# Autodesk Inventor assembly: OpenRaman.V1
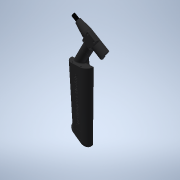
[picture p0: Inventor's stored thumbnail of the model, 180x180]
Saved by Autodesk Inventor 2020 (Build 240168000, 168)
## iProperties
Created: 2017-08-01
Part Number: OpenRaman.V1
Document SubType Name: Assembly
Designer: vmiguel
Author: vmiguel
## Documents named in this file (12)
- C:\Users\vmiguel\Documents\GitHub\OpenRaman\Hardware\OpenRaman.V1.iam
- C:\Users\vmiguel\Documents\GitHub\OpenRaman\Hardware\Supriments\TCD1304AP.ipt
- C:\Users\vmiguel\Documents\GitHub\OpenRaman\Hardware\PrismsGeometry.ipt
- C:\Users\vmiguel\Documents\GitHub\OpenRaman\Hardware\3D Printed Parts\SpectometerTube.ipt
- C:\Users\vmiguel\Documents\GitHub\OpenRaman\Hardware\3D Printed Parts\FirstPrismHolder.ipt
- C:\Users\vmiguel\Documents\GitHub\OpenRaman\Hardware\3D Printed Parts\PrismSensorHolder.ipt
- C:\Users\vmiguel\Documents\GitHub\OpenRaman\Hardware\Supriments\step_36396.ipt
- C:\Users\vmiguel\Documents\GitHub\OpenRaman\Hardware\Laser Cutted Parts\Slit.ipt
- C:\Users\vmiguel\Documents\GitHub\OpenRaman\Hardware\3D Printed Parts\NotchFilterScrew.ipt
- C:\Users\vmiguel\Documents\GitHub\OpenRaman\Hardware\3D Printed Parts\SpectoBoardCap.ipt
- C:\Users\vmiguel\Documents\GitHub\OpenRaman\Hardware\3D Printed Parts\RamanBody.ipt
- C:\Users\vmiguel\Documents\GitHub\OpenRaman\Hardware\Supriments\DPSSLaser.ipt
## Components (12 placed, 11 different names)
1. TCD1304AP:1 — Mate:3, Mate:4, Mate:5
2. PrismsGeometry:1 — Flush:2, Angle:1, Mate:1, Mate:2, Mate:3, Mate:4, Mate:5
3. SpectometerTube:1 — Flush:2, Angle:1, Mate:1, Flush:3, Flush:4
4. FirstPrismHolder:1 — Flush:3, Mate:2, Rotational:1, Mate:6, Mate:7, Flush:5, Rotational:3
5. PrismSensorHolder:1 — Flush:4, Flush:6
6. step_36396:1 — Rotational:1, Rotational:2
7. step_36396:2 — Rotational:2
8. Slit:1 — Mate:6, Mate:7
9. NotchFilterScrew:1 — Flush:5
10. SpectoBoardCap:1 — Flush:6
11. RamanBody:1 — Rotational:3, Rotational:4
12. DPSSLaser:1 — Rotational:4
## Relationships (17: Mate 7, Flush 5, RevoluteJoint 4, Angle 1)
- Flush:2: PrismsGeometry:1 ↔ SpectometerTube:1
- Angle:1 (-12 deg): PrismsGeometry:1 ↔ SpectometerTube:1
- Mate:1 (4 mm): PrismsGeometry:1 ↔ SpectometerTube:1
- Flush:3: SpectometerTube:1 ↔ FirstPrismHolder:1
- Mate:2: PrismsGeometry:1 ↔ FirstPrismHolder:1
- Mate:3: TCD1304AP:1 ↔ PrismsGeometry:1
- Mate:4: TCD1304AP:1 ↔ PrismsGeometry:1
- Mate:5: TCD1304AP:1 ↔ PrismsGeometry:1
- Flush:4: SpectometerTube:1 ↔ PrismSensorHolder:1
- Rotational:1 [RevoluteJoint]: FirstPrismHolder:1 ↔ step_36396:1
- Rotational:2 [RevoluteJoint] (15 mm): step_36396:1 ↔ step_36396:2
- Mate:6: FirstPrismHolder:1 ↔ Slit:1
- Mate:7: FirstPrismHolder:1 ↔ Slit:1
- Flush:5: FirstPrismHolder:1 ↔ NotchFilterScrew:1
- Flush:6: PrismSensorHolder:1 ↔ SpectoBoardCap:1
- Rotational:3 [RevoluteJoint]: FirstPrismHolder:1 ↔ RamanBody:1
- Rotational:4 [RevoluteJoint]: RamanBody:1 ↔ DPSSLaser:1
